# Autodesk Inventor assembly: BAcA_assembly
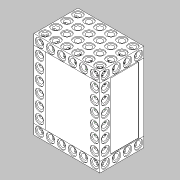
[picture p0: Inventor's stored thumbnail of the model, 180x180]
Saved by Autodesk Inventor 2019.3 (Build 233278000, 278)
## iProperties
Created: 2019-02-15
Part Number: BAcA_assembly
Document SubType Name: Assembly
Designer: Varga Daniel
Sending System: SolidWorks 2018
Last Author: david
Last Saved: 2019-02-15
Author: Varga Daniel
## Documents named in this file (4)
- C:\!_Dani\!_cloud\OneDrive\!_munka\Revolution\RevvyDemoKit\Structural parts\Demo parts\Battery\Inventor Imported\BAcA_assembly.iam
- C:\!_Dani\!_cloud\OneDrive\!_munka\Revolution\RevvyDemoKit\Structural parts\Demo parts\Battery\Inventor Imported\BAcA.ipt
- C:\!_Dani\!_cloud\OneDrive\!_munka\Revolution\RevvyDemoKit\Structural parts\Demo parts\Battery\Inventor Imported\Battery_holder_WZY-148-1_with_cable.iam
- C:\!_Dani\!_cloud\OneDrive\!_munka\Revolution\RevvyDemoKit\Structural parts\Demo parts\Battery\Inventor Imported\BAcA_3.ipt
## Components (3 placed, 3 different names)
1. BAcA:1 — Mate:3, Tangent:1, Angle:1, Angle:2, Mate:4, Flush:2, Flush:3
2. Battery_holder_WZY-148-1_with_cable:1 [sub-assembly] — Mate:3, Tangent:1, Angle:1, Tangent:2, Mate:4
3. BAcA_3:1 — Flush:2, Flush:3
## Relationships (8: Mate 2, Tangent 2, Angle 2, Flush 2)
- Mate:3: BAcA:1 ↔ Battery_holder_WZY-148-1_with_cable:1
- Tangent:1: BAcA:1 ↔ Battery_holder_WZY-148-1_with_cable:1
- Angle:1 (180 deg): BAcA:1 ↔ Battery_holder_WZY-148-1_with_cable:1
- Angle:2 (0 deg): BAcA:1
- Tangent:2: Battery_holder_WZY-148-1_with_cable:1
- Mate:4 (3.678 mm): BAcA:1 ↔ Battery_holder_WZY-148-1_with_cable:1
- Flush:2: BAcA:1 ↔ BAcA_3:1
- Flush:3: BAcA:1 ↔ BAcA_3:1
